# Autodesk Inventor assembly: PCB COMPLETA
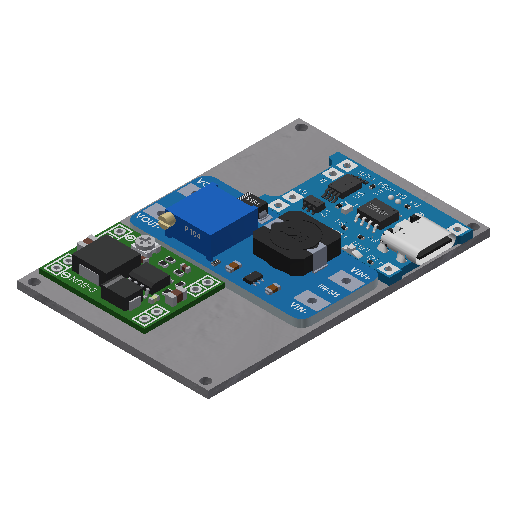
[picture p0: Inventor's stored thumbnail of the model, 512x512]
Saved by Autodesk Inventor 2025.2 (Build 292293000, 293)
## iProperties
Created: 2025-10-17
Part Number: PCB COMPLETA
Material: Generic
Document SubType Name: Assembly
Designer: Ricardo
Author: Ricardo
## Documents named in this file (6)
- C:\Users\Ricardo\Documents\Inventor\TFC\Componentes\d-sun-dc-dc-step-down-voltage-regulator-simple-version-1.snapshot.4\PCB COMPLETA.iam
- C:\Users\Ricardo\Documents\Inventor\TFC\Componentes\pcb sola.ipt
- C:\Users\Ricardo\Documents\Inventor\TFC\Componentes\tp4056-charging-module-2.snapshot.1\TP4056_Ens.iam
- C:\Users\Ricardo\Documents\Inventor\TFC\Componentes\mt3608-dc-to-dc-boost-converter-2-a-1.snapshot.4\MT3608 Converter\MT3608 Converter\MT3608 Converter_ens.iam
- C:\Users\Ricardo\Documents\Inventor\TFC\Componentes\d-sun-dc-dc-step-down-voltage-regulator-simple-version-1.snapshot.4\stepdown_en.iam
- C:\Users\Ricardo\Documents\Inventor\TFC\Componentes\female-header-pins-2.snapshot.2\HEADERS HEMBR.iam
## Components (6 placed, 5 different names)
1. pcb sola:1 — Mate:1, Flush:1, Flush:2, Mate:2, Flush:3, Mate:4, Flush:4, Mate:13, Mate:14, Flush:5, Mate:15, Flush:6
2. TP4056_Ens:1 [sub-assembly] — Mate:1, Flush:1, Flush:2, Mate:3
3. MT3608 Converter_ens:1 [sub-assembly] — Mate:2, Flush:3, Mate:3, Mate:5
4. stepdown_en:1 [sub-assembly] — Mate:4, Flush:4, Mate:5
5. HEADERS HEMBR:1 [sub-assembly] — Mate:13, Mate:14, Flush:5, Mate:16
6. HEADERS HEMBR:2 [sub-assembly] — Mate:15, Mate:16, Flush:6
## Relationships (15: Mate 9, Flush 6)
- Mate:1: pcb sola:1 ↔ TP4056_Ens:1
- Flush:1: pcb sola:1 ↔ TP4056_Ens:1
- Flush:2 (3.5 mm): pcb sola:1 ↔ TP4056_Ens:1
- Mate:2: pcb sola:1 ↔ MT3608 Converter_ens:1
- Flush:3 (1 mm): pcb sola:1 ↔ MT3608 Converter_ens:1
- Mate:3 (0.2 mm): TP4056_Ens:1 ↔ MT3608 Converter_ens:1
- Mate:4: pcb sola:1 ↔ stepdown_en:1
- Flush:4 (1 mm): pcb sola:1 ↔ stepdown_en:1
- Mate:5 (0.2 mm): MT3608 Converter_ens:1 ↔ stepdown_en:1
- Mate:13: pcb sola:1 ↔ HEADERS HEMBR:1
- Mate:14 (-5.5 mm): pcb sola:1 ↔ HEADERS HEMBR:1
- Flush:5 (13 mm): pcb sola:1 ↔ HEADERS HEMBR:1
- Mate:15: pcb sola:1 ↔ HEADERS HEMBR:2
- Mate:16 (23 mm): HEADERS HEMBR:1 ↔ HEADERS HEMBR:2
- Flush:6 (13 mm): pcb sola:1 ↔ HEADERS HEMBR:2
